# Autodesk Inventor assembly: RobotAlvaz
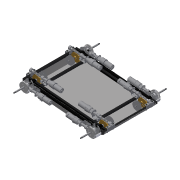
[picture p0: Inventor's stored thumbnail of the model, 180x180]
Saved by Autodesk Inventor 2015 SP1 (Build 190203100, 203)
## iProperties
Created: 2015-02-26
Part Number: RobotAlvaz
Document SubType Name: Assembly
Designer: laca
Author: laca
## Documents named in this file (5)
- C:\Users\laca\Desktop\Allamvizsga\Invntor\RobotMechanikaForMAtlabVer2\RobotAlvaz.iam
- C:\Users\laca\Desktop\Allamvizsga\Invntor\RobotMechanikaForMAtlabVer2\Lemez.ipt
- C:\Users\laca\Desktop\RobotMechanikaForMAtlabVer2\VizhutesVer2.iam
- C:\Users\laca\Desktop\RobotMechanikaForMAtlabVer2\VizPumpaVer2.ipt
- C:\Users\laca\Desktop\Allamvizsga\Invntor\RobotMechanikaForMAtlabVer2\FelAlvaz.ipt
## Components (5 placed, 4 different names)
1. FelAlvaz:3 — Flush:1, Mate:2, Mate:7
2. Lemez:1 — Flush:1, Mate:2, Mate:3, Mate:6, Mate:7
3. VizhutesVer2:1 [sub-assembly] — Mate:6, Flush:2
4. VizhutesVer2:2 [sub-assembly] — Mate:3, Flush:2
5. VizPumpaVer2:1
## Relationships (8: Mate 6, Flush 2)
- Flush:1: FelAlvaz:3 ↔ Lemez:1
- Mate:2: FelAlvaz:3 ↔ Lemez:1
- Mate:3: Lemez:1 ↔ VizhutesVer2:2
- [Mate] (70 mm): FelAlvaz:3 ↔ VizhutesVer2:2
- [Mate]: FelAlvaz:3 ↔ VizhutesVer2:2
- Mate:6: Lemez:1 ↔ VizhutesVer2:1
- Flush:2: VizhutesVer2:1 ↔ VizhutesVer2:2
- Mate:7: FelAlvaz:3 ↔ Lemez:1
